# Autodesk Inventor assembly: biggearsmallgearNOSPACER
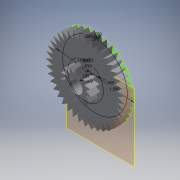
[picture p0: Inventor's stored thumbnail of the model, 180x180]
Saved by Autodesk Inventor 2018.3 (Build 223284000, 284)
## iProperties
Created: 2019-03-12
Part Number: biggearsmallgearNOSPACER
Document SubType Name: Assembly
Designer: F8PLTW
Author: F8PLTW
## Documents named in this file (3)
- D:\biggearsmallgearNOSPACER.iam
- D:\phonegearfinalBIG.ipt
- D:\phonecasegearSMALL.ipt
## Components (2 placed, 2 different names)
1. phonegearfinalBIG:1 — Mate:1, Mate:2
2. phonecasegearSMALL:1 — Mate:1, Mate:2
## Relationships (2: Mate 2)
- Mate:1: phonegearfinalBIG:1 ↔ phonecasegearSMALL:1
- Mate:2: phonegearfinalBIG:1 ↔ phonecasegearSMALL:1
